# Autodesk Inventor assembly: UEBG-Schuss
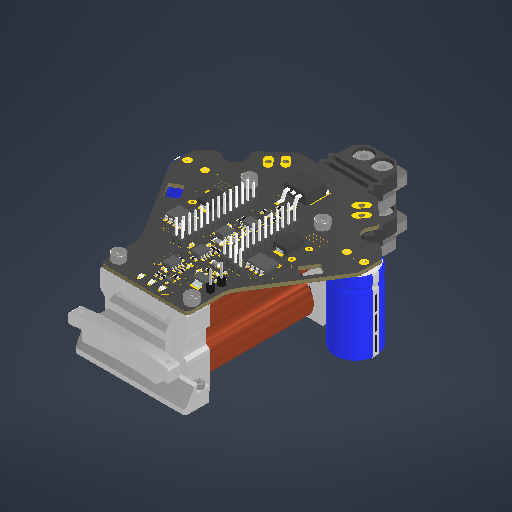
[picture p0: Inventor's stored thumbnail of the model, 512x512]
Saved by Autodesk Inventor 2025.2 (Build 292293000, 293)
## iProperties
Created: 2024-11-08
Part Number: UEBG-Schuss
Document SubType Name: Assembly
Designer: Fabian
Author: Fabian
## Documents named in this file (6)
- C:\Users\Faabs\Desktop\HBG v2025\Oberbaugruppen\OBG-Schuss\OBG-Schuss.iam
- C:\Users\Faabs\Desktop\HBG v2025\Unterbaugruppen\UBG-Schussbauteile\UBG-Schusskörper\UBG-Schusskörper.iam
- C:\Users\Faabs\Desktop\HBG v2025\Unterbaugruppen\UBG-Schussbauteile\UBG-Schuss\UBG-Schuss.iam
- C:\Users\Faabs\Desktop\HBG v2025\Unterbaugruppen\UBG-Schussbauteile\UBG-Hochschuss\UBG-Hochschuss.iam
- C:\Users\Faabs\Desktop\HBG v2025\Verbindungselemente\DIN 912\DIN 912 - M3 x 0,5 x 6 x 4,75.ipt
- C:\Users\Faabs\Desktop\HBG v2025\Platinen\Schussplatine\Schussplatine.ipt
## Components (8 placed, 5 different names)
1. UBG-Schusskörper:1 [sub-assembly] — Passend:6, Passend:7, Passend:8, Passend:9, Passend:10, Passend:11, Passend:12
2. UBG-Schuss:1 [sub-assembly] — Passend:10, Fluchtend:12, Passend:11
3. UBG-Hochschuss:1 [sub-assembly] — Passend:6, Fluchtend:13, Passend:12
4. Schussplatine:1 — Passend:7, Passend:8, Passend:9, Einfügen:1, Einfügen:2, Einfügen:3, Einfügen:4
5. DIN 912 - ersetzt durch DIN EN ISO 4762 M3 x 6:1 — Einfügen:2
6. DIN 912 - ersetzt durch DIN EN ISO 4762 M3 x 6:2 — Einfügen:1
7. DIN 912 - ersetzt durch DIN EN ISO 4762 M3 x 6:3 — Einfügen:3
8. DIN 912 - ersetzt durch DIN EN ISO 4762 M3 x 6:4 — Einfügen:4
## Relationships (13: Mate 7, Insert 4, Flush 2)
- Passend:6 [Mate]: UBG-Schusskörper:1 ↔ UBG-Hochschuss:1
- Passend:7 [Mate]: UBG-Schusskörper:1 ↔ Schussplatine:1
- Passend:8 [Mate]: UBG-Schusskörper:1 ↔ Schussplatine:1
- Passend:9 [Mate]: UBG-Schusskörper:1 ↔ Schussplatine:1
- Einfügen:1 [Insert]: Schussplatine:1 ↔ DIN 912 - ersetzt durch DIN EN ISO 4762 M3 x 6:2
- Einfügen:2 [Insert]: Schussplatine:1 ↔ DIN 912 - ersetzt durch DIN EN ISO 4762 M3 x 6:1
- Einfügen:3 [Insert]: Schussplatine:1 ↔ DIN 912 - ersetzt durch DIN EN ISO 4762 M3 x 6:3
- Einfügen:4 [Insert]: Schussplatine:1 ↔ DIN 912 - ersetzt durch DIN EN ISO 4762 M3 x 6:4
- Passend:10 [Mate]: UBG-Schusskörper:1 ↔ UBG-Schuss:1
- Fluchtend:12 [Flush]: UBG-Schuss:1
- Passend:11 [Mate] (0.05 mm): UBG-Schusskörper:1 ↔ UBG-Schuss:1
- Fluchtend:13 [Flush] (-12 mm): UBG-Hochschuss:1
- Passend:12 [Mate] (0.05 mm): UBG-Schusskörper:1 ↔ UBG-Hochschuss:1
